# Autodesk Inventor assembly: assemblage_nema8
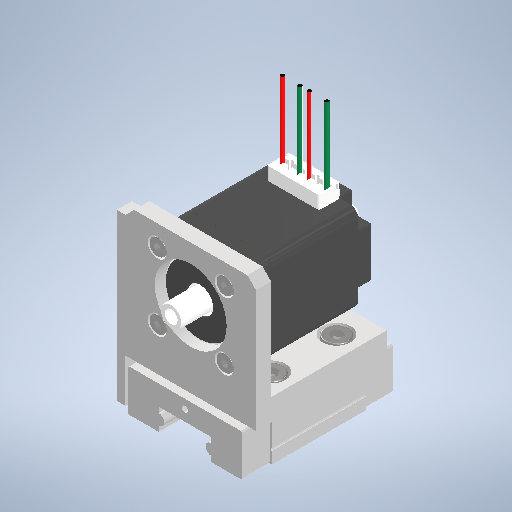
[picture p0: Inventor's stored thumbnail of the model, 512x512]
Saved by Autodesk Inventor 2025.1 (Build 291241000, 241)
## iProperties
Created: 2025-03-24
Part Number: assemblage_nema8
Document SubType Name: Assembly
Designer: felix
Author: felix
## Documents named in this file (6)
- D:\documents\projets inventor\Skibbidi Startech\assemblage_nema8.iam
- D:\documents\projets inventor\Skibbidi Startech\mgn12c_02.ipt
- D:\documents\projets inventor\Skibbidi Startech\support nema8.ipt
- C:\Users\felix\OneDrive - Haute Ecole de Namur-Liege-Luxembourg\Documents\Inventor\Content Center Files\R2025\fr-FR\BS EN ISO 4762\BS EN ISO 4762 - M3 x 10(1).ipt
- D:\documents\projets inventor\Skibbidi Startech\moteur_nema8.ipt
- C:\Users\felix\OneDrive - Haute Ecole de Namur-Liege-Luxembourg\Documents\Inventor\Content Center Files\R2025\fr-FR\BS EN ISO 4762\BS EN ISO 4762 - M2 x 5(1).ipt
## Components (11 placed, 5 different names)
1. mgn12c_02:1 — Placage:1, Placage:2, Placage:3
2. support nema8:1 — Placage:1, Placage:2, Placage:3, Rotation:1, Rotation:2, Rotation:3, Rotation:4, Placage:4, Placage:5, Placage:6, Placage:7, Placage:8, Placage:9, Placage:10, Placage:11, Placage:12, Placage:13, Placage:14
3. BS EN ISO 4762 : Pièce 1 Vis cylindrique à six pans creux - Métrique M3 x 10:1 — Rotation:4
4. BS EN ISO 4762 : Pièce 1 Vis cylindrique à six pans creux - Métrique M3 x 10:2 — Rotation:3
5. BS EN ISO 4762 : Pièce 1 Vis cylindrique à six pans creux - Métrique M3 x 10:3 — Rotation:2
6. BS EN ISO 4762 : Pièce 1 Vis cylindrique à six pans creux - Métrique M3 x 10:4 — Rotation:1
7. moteur_nema8:1 — Placage:4, Placage:5, Placage:6
8. BS EN ISO 4762 : Pièce 1 Vis cylindrique à six pans creux - Métrique M2 x 5:1 — Placage:13, Placage:14
9. BS EN ISO 4762 : Pièce 1 Vis cylindrique à six pans creux - Métrique M2 x 5:2 — Placage:11, Placage:12
10. BS EN ISO 4762 : Pièce 1 Vis cylindrique à six pans creux - Métrique M2 x 5:3 — Placage:9, Placage:10
11. BS EN ISO 4762 : Pièce 1 Vis cylindrique à six pans creux - Métrique M2 x 5:4 — Placage:7, Placage:8
## Relationships (18: Mate 14, RevoluteJoint 4)
- Placage:1 [Mate]: mgn12c_02:1 ↔ support nema8:1
- Placage:2 [Mate]: mgn12c_02:1 ↔ support nema8:1
- Placage:3 [Mate]: mgn12c_02:1 ↔ support nema8:1
- Rotation:1 [RevoluteJoint]: support nema8:1 ↔ BS EN ISO 4762 : Pièce 1 Vis cylindrique à six pans creux - Métrique M3 x 10:4
- Rotation:2 [RevoluteJoint]: support nema8:1 ↔ BS EN ISO 4762 : Pièce 1 Vis cylindrique à six pans creux - Métrique M3 x 10:3
- Rotation:3 [RevoluteJoint]: support nema8:1 ↔ BS EN ISO 4762 : Pièce 1 Vis cylindrique à six pans creux - Métrique M3 x 10:2
- Rotation:4 [RevoluteJoint]: support nema8:1 ↔ BS EN ISO 4762 : Pièce 1 Vis cylindrique à six pans creux - Métrique M3 x 10:1
- Placage:4 [Mate]: support nema8:1 ↔ moteur_nema8:1
- Placage:5 [Mate]: support nema8:1 ↔ moteur_nema8:1
- Placage:6 [Mate]: support nema8:1 ↔ moteur_nema8:1
- Placage:7 [Mate]: support nema8:1 ↔ BS EN ISO 4762 : Pièce 1 Vis cylindrique à six pans creux - Métrique M2 x 5:4
- Placage:8 [Mate]: support nema8:1 ↔ BS EN ISO 4762 : Pièce 1 Vis cylindrique à six pans creux - Métrique M2 x 5:4
- Placage:9 [Mate]: support nema8:1 ↔ BS EN ISO 4762 : Pièce 1 Vis cylindrique à six pans creux - Métrique M2 x 5:3
- Placage:10 [Mate]: support nema8:1 ↔ BS EN ISO 4762 : Pièce 1 Vis cylindrique à six pans creux - Métrique M2 x 5:3
- Placage:11 [Mate]: support nema8:1 ↔ BS EN ISO 4762 : Pièce 1 Vis cylindrique à six pans creux - Métrique M2 x 5:2
- Placage:12 [Mate]: support nema8:1 ↔ BS EN ISO 4762 : Pièce 1 Vis cylindrique à six pans creux - Métrique M2 x 5:2
- Placage:13 [Mate]: support nema8:1 ↔ BS EN ISO 4762 : Pièce 1 Vis cylindrique à six pans creux - Métrique M2 x 5:1
- Placage:14 [Mate]: support nema8:1 ↔ BS EN ISO 4762 : Pièce 1 Vis cylindrique à six pans creux - Métrique M2 x 5:1
